# Autodesk Inventor assembly: TrussCC_testasm
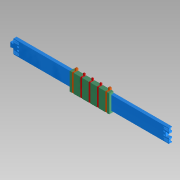
[picture p0: Inventor's stored thumbnail of the model, 180x180]
Saved by Autodesk Inventor 2021 (Build 250183000, 183)
## iProperties
Created: 2021-02-11
Part Number: TrussCC_testasm
Document SubType Name: Assembly
Designer: kumagai
Author: kumagai
## Documents named in this file (6)
- X:\Develop\CAD\PlaRails\TrussCC\TrussCC_testasm.iam
- X:\Develop\CAD\PlaRails\TrussCC\TrussCC_box.ipt
- X:\Develop\CAD\PlaRails\TrussCC\TrussCC_S1.ipt
- X:\Develop\CAD\PlaRails\TrussCC\TrussCC_S2.ipt
- X:\Develop\CAD\PlaRails\StraightRail\StraightRail_i\StraightMF215.iam
- X:\Develop\CAD\PlaRails\StraightRail\StraightRail_i.iam
## Components (8 placed, 4 different names)
1. TrussCC_box:1 — フラッシュ:4, フラッシュ:5, メイト:3, メイト:7, フラッシュ:7, フラッシュ:8, メイト:9, メイト:10
2. StraightMF215:1 [sub-assembly] — フラッシュ:9, フラッシュ:10, メイト:8, メイト:10
3. StraightMF215:2 [sub-assembly] — フラッシュ:9, フラッシュ:10, メイト:8, メイト:9
4. TrussCC_S1:1 — フラッシュ:4, フラッシュ:5, メイト:3
5. TrussCC_S1:2
6. TrussCC_S1:3
7. TrussCC_S2:1 — メイト:7, フラッシュ:7, フラッシュ:8
8. TrussCC_S2:2
## Component patterns: (3 elements, first: TrussCC_S1:1), (2 elements, first: TrussCC_S2:1)
## Relationships (11: Flush 6, Mate 5)
- フラッシュ:4 [Flush]: TrussCC_box:1 ↔ TrussCC_S1:1
- フラッシュ:5 [Flush]: TrussCC_box:1 ↔ TrussCC_S1:1
- メイト:3 [Mate]: TrussCC_box:1 ↔ TrussCC_S1:1
- メイト:7 [Mate]: TrussCC_box:1 ↔ TrussCC_S2:1
- フラッシュ:7 [Flush]: TrussCC_box:1 ↔ TrussCC_S2:1
- フラッシュ:8 [Flush] (46 mm): TrussCC_box:1 ↔ TrussCC_S2:1
- フラッシュ:9 [Flush]: StraightMF215:1 ↔ StraightMF215:2
- フラッシュ:10 [Flush]: StraightMF215:1 ↔ StraightMF215:2
- メイト:8 [Mate]: StraightMF215:1 ↔ StraightMF215:2
- メイト:9 [Mate]: TrussCC_box:1 ↔ StraightMF215:2
- メイト:10 [Mate]: TrussCC_box:1 ↔ StraightMF215:1
